# Autodesk Inventor assembly: X-Gantry Joiner Right V4 Assembly
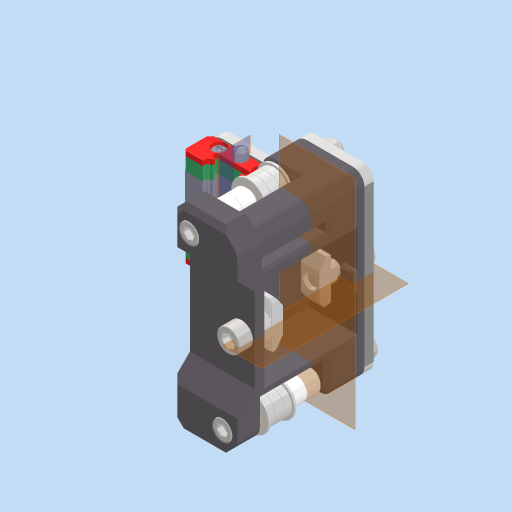
[picture p0: Inventor's stored thumbnail of the model, 512x512]
Saved by Autodesk Inventor 2023.2 (Build 272271000, 271)
## iProperties
Created: 2024-02-08
Part Number: X-Gantry Joiner Right V4 Assembly
Document SubType Name: Assembly
Designer: Nils Bade
Author: Nils Bade
## Documents named in this file (14)
- C:\Users\nilsb\Documents\Inventor\Projektarbeit-Bade\RatRig_Bade\X-Gantry Joiner Right V4 Assembly.iam
- C:\Users\nilsb\Documents\Inventor\Projektarbeit-Bade\RatRig_modified\xy Joiner Right for 4040 V3.ipt
- C:\Users\nilsb\Documents\Inventor\Projektarbeit-Bade\RatRig_modified\XY Joiner Plate for 4040 V3.ipt
- C:\Users\nilsb\Documents\Inventor\Projektarbeit-Bade\RatRig_modified\MGN15 Linear-Rail-Block.ipt
- C:\Users\nilsb\Documents\Inventor\Projektarbeit-Bade\Schrauben\Cap Head Screw M6x12 v2.ipt
- C:\Users\nilsb\Documents\Inventor\Projektarbeit-Bade\Schrauben\Cap Head Screw M6x16.ipt
- C:\Users\nilsb\Documents\Inventor\Projektarbeit-Bade\RatRig_modified\T-NUT - DropIn 4040 SERIES - M6.ipt
- C:\Users\nilsb\Documents\Inventor\Projektarbeit-Bade\Schrauben\Cap Head Screw M5x60.ipt
- C:\Users\nilsb\Documents\Inventor\Projektarbeit-Bade\RatRig_Standards\Hex Locking Nut - M5 v2.ipt
- C:\Users\nilsb\Documents\Inventor\Projektarbeit-Bade\RatRig_Standards\Mini Precision Shim - 8x5x1mm v2.ipt
- C:\Users\nilsb\Documents\Inventor\Projektarbeit-Bade\RatRig_Standards\Ball Bearing - F695ZZ v1.ipt
- C:\Users\nilsb\Documents\Inventor\Projektarbeit-Bade\RatRig_Standards\Ball Bearing - 695ZZ v1.ipt
- C:\Users\nilsb\Documents\Inventor\Projektarbeit-Bade\RatRig_Standards\Aluminium Spacer - 6mm v2.ipt
- C:\Users\nilsb\Documents\Inventor\Projektarbeit-Bade\Schrauben\Cap Head Screw M3x8 v2.ipt
## Components (31 placed, 13 different names)
1. xy Joiner Right for 4040 V3:1 — Passend:1, Passend:2, Passend:3, Passend:8, Passend:10, Winkel:1, Winkel:2, Passend:13, Passend:14, Passend:56, Passend:57, Passend:58, Passend:59, Passend:61, Passend:62
2. XY Joiner Plate for 4040 V3:1 — Passend:1, Passend:2, Passend:3, Passend:4, Passend:5, Passend:6, Passend:7, Passend:9, Passend:55, Passend:60
3. MGN15 Linear-Rail-Block:1 — Passend:4, Passend:5, Passend:6
4. Cap Head Screw M3x8 v2:1
5. Cap Head Screw M3x8 v2:2
6. Cap Head Screw M3x8 v2:3
7. Cap Head Screw M3x8 v2:4
8. Cap Head Screw M6x12 v2:1 — Passend:8, Passend:10, Passend:12
9. Cap Head Screw M6x16:1 — Passend:7, Passend:9, Passend:11
10. T-NUT - DROP IN TYPE FOR 40 SERIES - M6:1 — Passend:12, Winkel:2, Passend:14
11. T-NUT - DROP IN TYPE FOR 40 SERIES - M6:2 — Passend:11, Winkel:1, Passend:13
12. Cap Head Screw M5x60:1 — Passend:59, Passend:62
13. Hex Locking Nut - M5 v2:1 — Passend:60
14. Mini Precision Shim - 8x5x1mm v2:1
15. Mini Precision Shim - 8x5x1mm v2:2
16. Mini Precision Shim - 8x5x1mm v2:3 — Passend:61
17. Ball Bearing - F695ZZ v1:1
18. Ball Bearing - F695ZZ v1:2
19. Ball Bearing - 695ZZ v1:1
20. Aluminium Spacer - 6mm v2:1
21. Aluminium Spacer - 6mm v2:2
22. Cap Head Screw M5x60:2 — Passend:56, Passend:58
23. Hex Locking Nut - M5 v2:2 — Passend:55
24. Mini Precision Shim - 8x5x1mm v2:4
25. Mini Precision Shim - 8x5x1mm v2:5
26. Mini Precision Shim - 8x5x1mm v2:6 — Passend:57
27. Ball Bearing - F695ZZ v1:3
28. Ball Bearing - F695ZZ v1:4
29. Ball Bearing - 695ZZ v1:2
30. Aluminium Spacer - 6mm v2:3
31. Aluminium Spacer - 6mm v2:4
## Relationships (64: Mate 62, Angle 2)
- Passend:1 [Mate]: xy Joiner Right for 4040 V3:1 ↔ XY Joiner Plate for 4040 V3:1
- Passend:2 [Mate]: xy Joiner Right for 4040 V3:1 ↔ XY Joiner Plate for 4040 V3:1
- Passend:3 [Mate]: xy Joiner Right for 4040 V3:1 ↔ XY Joiner Plate for 4040 V3:1
- Passend:4 [Mate]: XY Joiner Plate for 4040 V3:1 ↔ MGN15 Linear-Rail-Block:1
- Passend:5 [Mate]: XY Joiner Plate for 4040 V3:1 ↔ MGN15 Linear-Rail-Block:1
- Passend:6 [Mate]: XY Joiner Plate for 4040 V3:1 ↔ MGN15 Linear-Rail-Block:1
- Passend:7 [Mate]: XY Joiner Plate for 4040 V3:1 ↔ Cap Head Screw M6x16:1
- Passend:8 [Mate]: xy Joiner Right for 4040 V3:1 ↔ Cap Head Screw M6x12 v2:1
- Passend:9 [Mate]: XY Joiner Plate for 4040 V3:1 ↔ Cap Head Screw M6x16:1
- Passend:10 [Mate]: xy Joiner Right for 4040 V3:1 ↔ Cap Head Screw M6x12 v2:1
- Passend:11 [Mate]: Cap Head Screw M6x16:1 ↔ T-NUT - DROP IN TYPE FOR 40 SERIES - M6:2
- Passend:12 [Mate]: Cap Head Screw M6x12 v2:1 ↔ T-NUT - DROP IN TYPE FOR 40 SERIES - M6:1
- Winkel:1 [Angle] (0 deg): xy Joiner Right for 4040 V3:1 ↔ T-NUT - DROP IN TYPE FOR 40 SERIES - M6:2
- Winkel:2 [Angle] (0 deg): xy Joiner Right for 4040 V3:1 ↔ T-NUT - DROP IN TYPE FOR 40 SERIES - M6:1
- Passend:13 [Mate] (5.5 mm): xy Joiner Right for 4040 V3:1 ↔ T-NUT - DROP IN TYPE FOR 40 SERIES - M6:2
- Passend:14 [Mate] (4.6 mm): xy Joiner Right for 4040 V3:1 ↔ T-NUT - DROP IN TYPE FOR 40 SERIES - M6:1
- [Mate]: XY Joiner Plate for 4040 V3:1 ↔ Cap Head Screw M3x8 v2:4
- [Mate]: XY Joiner Plate for 4040 V3:1 ↔ Cap Head Screw M3x8 v2:1
- [Mate]: XY Joiner Plate for 4040 V3:1 ↔ Cap Head Screw M3x8 v2:2
- [Mate]: XY Joiner Plate for 4040 V3:1 ↔ Cap Head Screw M3x8 v2:3
- [Mate]: XY Joiner Plate for 4040 V3:1 ↔ Cap Head Screw M3x8 v2:4
- [Mate]: XY Joiner Plate for 4040 V3:1 ↔ Cap Head Screw M3x8 v2:1
- [Mate]: XY Joiner Plate for 4040 V3:1 ↔ Cap Head Screw M3x8 v2:2
- [Mate]: XY Joiner Plate for 4040 V3:1 ↔ Cap Head Screw M3x8 v2:3
- [Mate]: Cap Head Screw M5x60:1 ↔ Hex Locking Nut - M5 v2:1
- [Mate]: Cap Head Screw M5x60:1 ↔ Mini Precision Shim - 8x5x1mm v2:1
- [Mate]: Cap Head Screw M5x60:1 ↔ Ball Bearing - F695ZZ v1:1
- [Mate]: Mini Precision Shim - 8x5x1mm v2:1 ↔ Ball Bearing - F695ZZ v1:1
- [Mate]: Cap Head Screw M5x60:1 ↔ Ball Bearing - 695ZZ v1:1
- [Mate]: Ball Bearing - F695ZZ v1:1 ↔ Ball Bearing - 695ZZ v1:1
- [Mate]: Cap Head Screw M5x60:1 ↔ Ball Bearing - F695ZZ v1:2
- [Mate]: Ball Bearing - F695ZZ v1:2 ↔ Ball Bearing - 695ZZ v1:1
- [Mate]: Cap Head Screw M5x60:1 ↔ Mini Precision Shim - 8x5x1mm v2:2
- [Mate]: Mini Precision Shim - 8x5x1mm v2:2 ↔ Ball Bearing - F695ZZ v1:2
- [Mate]: Cap Head Screw M5x60:1 ↔ Aluminium Spacer - 6mm v2:1
- [Mate]: Mini Precision Shim - 8x5x1mm v2:2 ↔ Aluminium Spacer - 6mm v2:1
- [Mate]: Cap Head Screw M5x60:1 ↔ Aluminium Spacer - 6mm v2:2
- [Mate]: Aluminium Spacer - 6mm v2:1 ↔ Aluminium Spacer - 6mm v2:2
- [Mate]: Cap Head Screw M5x60:1 ↔ Mini Precision Shim - 8x5x1mm v2:3
- [Mate]: Mini Precision Shim - 8x5x1mm v2:3 ↔ Aluminium Spacer - 6mm v2:2
- [Mate]: Cap Head Screw M5x60:2 ↔ Hex Locking Nut - M5 v2:2
- [Mate]: Cap Head Screw M5x60:2 ↔ Mini Precision Shim - 8x5x1mm v2:6
- [Mate]: Cap Head Screw M5x60:2 ↔ Ball Bearing - F695ZZ v1:4
- [Mate]: Mini Precision Shim - 8x5x1mm v2:6 ↔ Ball Bearing - F695ZZ v1:4
- [Mate]: Cap Head Screw M5x60:2 ↔ Ball Bearing - 695ZZ v1:2
- [Mate]: Ball Bearing - F695ZZ v1:4 ↔ Ball Bearing - 695ZZ v1:2
- [Mate]: Cap Head Screw M5x60:2 ↔ Ball Bearing - F695ZZ v1:3
- [Mate]: Ball Bearing - F695ZZ v1:3 ↔ Ball Bearing - 695ZZ v1:2
- [Mate]: Cap Head Screw M5x60:2 ↔ Mini Precision Shim - 8x5x1mm v2:5
- [Mate]: Mini Precision Shim - 8x5x1mm v2:5 ↔ Ball Bearing - F695ZZ v1:3
- [Mate]: Cap Head Screw M5x60:2 ↔ Aluminium Spacer - 6mm v2:3
- [Mate]: Mini Precision Shim - 8x5x1mm v2:5 ↔ Aluminium Spacer - 6mm v2:3
- [Mate]: Cap Head Screw M5x60:2 ↔ Aluminium Spacer - 6mm v2:4
- [Mate]: Aluminium Spacer - 6mm v2:3 ↔ Aluminium Spacer - 6mm v2:4
- [Mate]: Cap Head Screw M5x60:2 ↔ Mini Precision Shim - 8x5x1mm v2:4
- [Mate]: Mini Precision Shim - 8x5x1mm v2:4 ↔ Aluminium Spacer - 6mm v2:4
- Passend:55 [Mate]: XY Joiner Plate for 4040 V3:1 ↔ Hex Locking Nut - M5 v2:2
- Passend:56 [Mate]: xy Joiner Right for 4040 V3:1 ↔ Cap Head Screw M5x60:2
- Passend:57 [Mate]: xy Joiner Right for 4040 V3:1 ↔ Mini Precision Shim - 8x5x1mm v2:6
- Passend:58 [Mate]: xy Joiner Right for 4040 V3:1 ↔ Cap Head Screw M5x60:2
- Passend:59 [Mate]: xy Joiner Right for 4040 V3:1 ↔ Cap Head Screw M5x60:1
- Passend:60 [Mate]: XY Joiner Plate for 4040 V3:1 ↔ Hex Locking Nut - M5 v2:1
- Passend:61 [Mate]: xy Joiner Right for 4040 V3:1 ↔ Mini Precision Shim - 8x5x1mm v2:3
- Passend:62 [Mate]: xy Joiner Right for 4040 V3:1 ↔ Cap Head Screw M5x60:1
## Named parameters: d5_d37 = 0 mm, d8_d40 = 0 mm, d9_d42 = 0 mm, d10_d43 = 0 mm, d11_d44 = 0 mm
